# Autodesk Inventor assembly: HGH20CA1R250Z0H_FILE_1
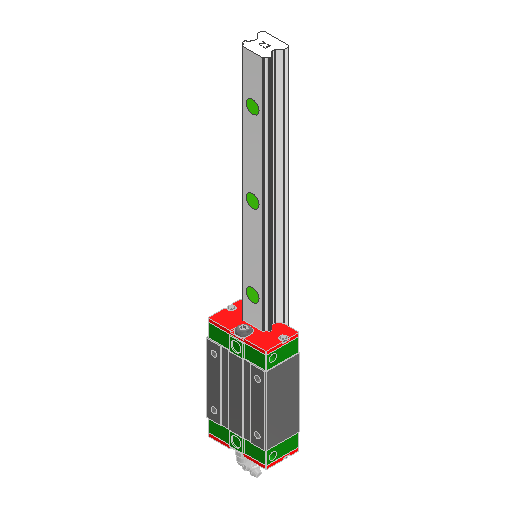
[picture p0: Inventor's stored thumbnail of the model, 512x512]
Saved by Autodesk Inventor 2024.3 (Build 283343000, 343)
## iProperties
Created: 2025-06-08
Part Number: HGH20CA1R250Z0H_FILE_1
Document SubType Name: Assembly
Designer: MPA
Part Number: HGH20CA1R250Z0H_FILE
Revision: NONE
Author: HIWIN GmbH
Title: cctmp_E6CB3DAF-07BE-41EC-A39F-681FA4047524_2025_06_08_12_44_05_0798_34176..stp
Organization: CADClick - www.CADClick.com
Description: STEP AP214
Authorization: unknown authorization
Preprocessor: Spatial InterOp 3D
Author: MPA
## Documents named in this file (3)
- C:\MPA - shortPath\magisterka\V3\Workspace\Zakupowe\hiwin\HGH20CA1R250Z0H_FILE_1\HGH20CA1R250Z0H_FILE_1\HGH20CA1R250Z0H_FILE_1.iam
- C:\MPA - shortPath\magisterka\V3\Workspace\Zakupowe\hiwin\HGH20CA1R250Z0H_FILE_1\HGH20CA1R250Z0H_FILE_1\2025_06_08_12_44_05_0798.ipt
- C:\MPA - shortPath\magisterka\V3\Workspace\Zakupowe\hiwin\HGH20CA1R250Z0H_FILE_1\HGH20CA1R250Z0H_FILE_1\2025_06_08_12_44_05_0783.ipt
## Components (2 placed, 2 different names)
1. 2025_06_08_12_44_05_0798 — Mate:1, Mate:2
2. 2025_06_08_12_44_05_0783 — Flush:1, Flush:2, Flush:3, Mate:1, Mate:2
## Relationships (5: Flush 3, Mate 2)
- Flush:1: 2025_06_08_12_44_05_0783
- Flush:2: 2025_06_08_12_44_05_0783
- Flush:3: 2025_06_08_12_44_05_0783
- Mate:1: 2025_06_08_12_44_05_0798 ↔ 2025_06_08_12_44_05_0783
- Mate:2: 2025_06_08_12_44_05_0798 ↔ 2025_06_08_12_44_05_0783
